# Autodesk Inventor assembly: montagem final Mars Rover
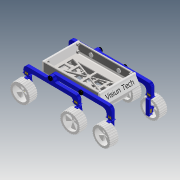
[picture p0: Inventor's stored thumbnail of the model, 180x180]
Saved by Autodesk Inventor 2021 (Build 250183000, 183)
## iProperties
Created: 2020-11-19
Part Number: montagem final Mars Rover
Document SubType Name: Assembly
Designer: evert
Author: evert
## Documents named in this file (16)
- C:\Users\evert\OneDrive\Área de Trabalho\novo mars\montagem final Mars Rover.iam
- C:\Users\evert\OneDrive\Área de Trabalho\novo mars\chassi.ipt
- C:\Users\evert\OneDrive\Área de Trabalho\novo mars\motor frente.ipt
- C:\Users\evert\OneDrive\Área de Trabalho\novo mars\suporte.ipt
- C:\Users\evert\OneDrive\Área de Trabalho\novo mars\sup para 2 motor.ipt
- C:\Users\evert\OneDrive\Área de Trabalho\novo mars\motor roda.ipt
- C:\Users\evert\OneDrive\Área de Trabalho\novo mars\roda.ipt
- C:\Users\evert\OneDrive\Área de Trabalho\novo mars\SG90 - Micro Servo 9g - Tower Pro.1_MIR.ipt
- C:\Users\evert\OneDrive\Área de Trabalho\novo mars\sup para 2 motor_MIR.ipt
- C:\Users\evert\OneDrive\Área de Trabalho\novo mars\motor roda_MIR.ipt
- C:\Users\evert\OneDrive\Área de Trabalho\novo mars\roda_MIR.ipt
- C:\Users\evert\OneDrive\Área de Trabalho\novo mars\sup frontal.ipt
- C:\Users\evert\OneDrive\Área de Trabalho\novo mars\tamp sup frontal.ipt
- C:\Users\evert\OneDrive\Área de Trabalho\novo mars\tampa frontal mars.ipt
- C:\Users\evert\OneDrive\Área de Trabalho\novo mars\tampa parte de traz mars.ipt
- C:\Users\evert\OneDrive\Área de Trabalho\novo mars\SG90 - Micro Servo 9g.ipt
## Components (29 placed, 15 different names)
1. chassi:1 — Coincidente:1, Ângulo:1, Rotativa:21, Rígida:4, Rotativa:23, Rotativa:25, Rígida:5, Rígida:6
2. motor frente:1 — Rotativa:6
3. sup para 2 motor:1 — Rotativa:7, Rígida:7
4. motor roda:1 — Rotativa:6, Rotativa:9
5. motor roda:2 — Rotativa:7, Rotativa:10
6. motor roda:3 — Rotativa:11
7. roda:1 — Rotativa:9
8. roda:2 — Rotativa:10
9. roda:3 — Rotativa:11
10. SG90 - Micro Servo 9g - Tower Pro.1_MIR:1 — Rotativa:15
11. sup para 2 motor_MIR:1 — Rotativa:16, Rígida:8
12. motor roda_MIR:1 — Rotativa:15, Rotativa:18
13. motor roda_MIR:2 — Rotativa:16, Rotativa:19
14. motor roda_MIR:3 — Rotativa:20
15. roda_MIR:1 — Rotativa:18
16. roda_MIR:2 — Rotativa:19
17. roda_MIR:3 — Rotativa:20
18. sup frontal:1 — Rotativa:21, Rígida:3
19. tamp sup frontal:1 — Rígida:3
20. tamp sup frontal:2 — Rotativa:22
21. sup frontal:2 — Rígida:4, Rotativa:22
22. suporte:1 — Rotativa:23, Rotativa:24
23. tamp sup frontal:3 — Rotativa:24
24. suporte:2 — Rotativa:25, Rotativa:26
25. tamp sup frontal:4 — Rotativa:26
26. tampa frontal mars:1 — Rígida:5
27. tampa parte de traz mars:1 — Rígida:6
28. SG90 - Micro Servo 9g:1 — Rígida:7
29. SG90 - Micro Servo 9g:2 — Rígida:8
## Relationships (24: RevoluteJoint 16, WeldJoint 6, Mate 1, Angle 1)
- Rotativa:6 [RevoluteJoint]: motor frente:1 ↔ motor roda:1
- Rotativa:7 [RevoluteJoint]: sup para 2 motor:1 ↔ motor roda:2
- Rotativa:9 [RevoluteJoint]: motor roda:1 ↔ roda:1
- Rotativa:10 [RevoluteJoint]: motor roda:2 ↔ roda:2
- Rotativa:11 [RevoluteJoint]: motor roda:3 ↔ roda:3
- Coincidente:1 [Mate]: chassi:1
- Ângulo:1 [Angle] (0 deg): chassi:1
- Rotativa:15 [RevoluteJoint]: SG90 - Micro Servo 9g - Tower Pro.1_MIR:1 ↔ motor roda_MIR:1
- Rotativa:16 [RevoluteJoint]: sup para 2 motor_MIR:1 ↔ motor roda_MIR:2
- Rotativa:18 [RevoluteJoint]: motor roda_MIR:1 ↔ roda_MIR:1
- Rotativa:19 [RevoluteJoint]: motor roda_MIR:2 ↔ roda_MIR:2
- Rotativa:20 [RevoluteJoint]: motor roda_MIR:3 ↔ roda_MIR:3
- Rotativa:21 [RevoluteJoint]: chassi:1 ↔ sup frontal:1
- Rígida:3 [WeldJoint]: sup frontal:1 ↔ tamp sup frontal:1
- Rígida:4 [WeldJoint]: chassi:1 ↔ sup frontal:2
- Rotativa:22 [RevoluteJoint] (1.5875 mm): tamp sup frontal:2 ↔ sup frontal:2
- Rotativa:23 [RevoluteJoint]: chassi:1 ↔ suporte:1
- Rotativa:24 [RevoluteJoint]: suporte:1 ↔ tamp sup frontal:3
- Rotativa:25 [RevoluteJoint]: chassi:1 ↔ suporte:2
- Rotativa:26 [RevoluteJoint]: suporte:2 ↔ tamp sup frontal:4
- Rígida:5 [WeldJoint]: chassi:1 ↔ tampa frontal mars:1
- Rígida:6 [WeldJoint]: chassi:1 ↔ tampa parte de traz mars:1
- Rígida:7 [WeldJoint]: sup para 2 motor:1 ↔ SG90 - Micro Servo 9g:1
- Rígida:8 [WeldJoint]: sup para 2 motor_MIR:1 ↔ SG90 - Micro Servo 9g:2
